# Autodesk Inventor assembly: inner
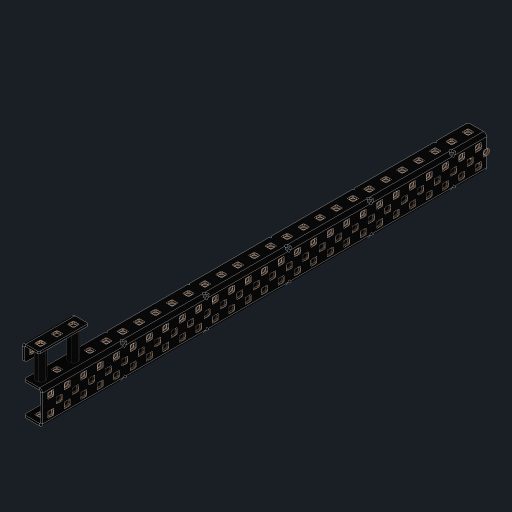
[picture p0: Inventor's stored thumbnail of the model, 512x512]
Saved by Autodesk Inventor 2024 (Build 280153000, 153)
## iProperties
Created: 2024-03-09
Part Number: inner
Document SubType Name: Assembly
Designer: Averey Ku
Author: Averey Ku
## Documents named in this file (5)
- D:\vex_robotics\hardware\cad\eca\chassis\drivebay\inner.iam
- D:\vex_robotics\hardware\cad\VEX-CAD-Inventor-1.41\Structure\C Channel\Aluminum 1x2x1\Alu C 1x2x1x27.ipt
- D:\vex_robotics\hardware\cad\VEX-CAD-Inventor-1.41\Structure\Standoff\Standoff .875.ipt
- D:\vex_robotics\hardware\cad\VEX-CAD-Inventor-1.41\Structure\Standoff.ipt
- D:\vex_robotics\hardware\cad\VEX-CAD-Inventor-1.41\Structure\Angle\Aluminum 1x1\Alu Angle 1x1x3.ipt
## Components (4 placed, 3 different names)
1. Alu C 1x2x1x27:1 — Insert:1, Insert:2
2. Standoff .875:1 — Insert:1, Insert:3
3. Standoff .875:2 — Insert:2, Mate:1
4. Alu Angle 1x1x3:1 — Insert:3, Mate:1
## Relationships (4: Insert 3, Mate 1)
- Insert:1: Alu C 1x2x1x27:1 ↔ Standoff .875:1
- Insert:2: Alu C 1x2x1x27:1 ↔ Standoff .875:2
- Insert:3: Standoff .875:1 ↔ Alu Angle 1x1x3:1
- Mate:1: Standoff .875:2 ↔ Alu Angle 1x1x3:1
